# Autodesk Inventor assembly: Motor_ra8846s
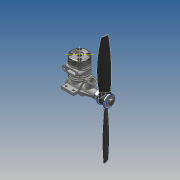
[picture p0: Inventor's stored thumbnail of the model, 180x180]
Saved by Autodesk Inventor 2021 (Build 250183000, 183)
## iProperties
Created: 2021-01-14
Part Number: Motor_ra8846s
Document SubType Name: Assembly
Designer: Sander
Author: Sander
## Documents named in this file (17)
- C:\Users\ricar\OneDrive - Fachhochschule Aachen\Mechatronik I\CAD\INVENTOR\Proyectos\Daten\Motor_ra8846s.iam
- C:\Users\ricar\OneDrive - Fachhochschule Aachen\Mechatronik I\CAD\INVENTOR\Proyectos\Daten\Motorblock_ra8846s.ipt
- C:\Users\ricar\OneDrive - Fachhochschule Aachen\Mechatronik I\CAD\INVENTOR\Proyectos\Daten\Zylinderkopf_ra8846s.ipt
- C:\Users\ricar\OneDrive - Fachhochschule Aachen\Mechatronik I\CAD\INVENTOR\Proyectos\Daten\Gehäusedeckel_ra8846s.ipt
- C:\Users\ricar\OneDrive - Fachhochschule Aachen\Mechatronik I\CAD\INVENTOR\Proyectos\Daten\Zylinderbuchse_ra8846s.ipt
- C:\Users\ricar\OneDrive - Fachhochschule Aachen\Mechatronik I\CAD\INVENTOR\Proyectos\Daten\Zylinderbuchsenring_ra8846s.ipt
- C:\Users\ricar\OneDrive - Fachhochschule Aachen\Mechatronik I\CAD\INVENTOR\Proyectos\Daten\Schlitzschraube_ra8846s\Schlitzschraube_ra8846s-01.ipt
- C:\Users\ricar\OneDrive - Fachhochschule Aachen\Mechatronik I\CAD\INVENTOR\Proyectos\Daten\Schlitzschraube_ra8846s.ipt
- C:\Users\ricar\OneDrive - Fachhochschule Aachen\Mechatronik I\CAD\INVENTOR\Proyectos\Daten\Unterlegescheibe_ra8846s.ipt
- C:\Users\ricar\OneDrive - Fachhochschule Aachen\Mechatronik I\CAD\INVENTOR\Proyectos\Daten\Kurbelwelle_ra8846s.ipt
- C:\Users\ricar\OneDrive - Fachhochschule Aachen\Mechatronik I\CAD\INVENTOR\Proyectos\Daten\Kolben_ra8846s.ipt
- C:\Users\ricar\OneDrive - Fachhochschule Aachen\Mechatronik I\CAD\INVENTOR\Proyectos\Daten\Kolbenbolzen_ra8846s.ipt
- C:\Users\ricar\OneDrive - Fachhochschule Aachen\Mechatronik I\CAD\INVENTOR\Proyectos\Daten\Pleuel_ra8846s.ipt
- C:\Users\ricar\OneDrive - Fachhochschule Aachen\Mechatronik I\CAD\INVENTOR\Proyectos\Daten\Propellernabe_ra8846s.ipt
- C:\Users\ricar\OneDrive - Fachhochschule Aachen\Mechatronik I\CAD\INVENTOR\Proyectos\Daten\propeller_ra8846s.ipt
- C:\Users\ricar\OneDrive - Fachhochschule Aachen\Mechatronik I\CAD\INVENTOR\Proyectos\Daten\Propellerscheib_ra8846s.ipt
- C:\Users\ricar\OneDrive - Fachhochschule Aachen\Mechatronik I\CAD\INVENTOR\Proyectos\Daten\Sechskantenschraube_ra8846s.ipt
## Components (18 placed, 15 different names)
1. Motorblock_ra8846s:1 — Einfügen:1, Einfügen:2, Einfügen:3, Einfügen:4, Einfügen:6, Einfügen:8
2. Zylinderkopf_ra8846s:1 — Einfügen:1, Einfügen:5
3. Gehäusedeckel_ra8846s:1 — Einfügen:2
4. Zylinderbuchse_ra8846s:1 — Einfügen:3, Passend:3
5. Zylinderbuchsenring_ra8846s:1 — Einfügen:4
6. Unterlegescheibe_ra8846s:1 — Einfügen:6, Einfügen:7
7. Kurbelwelle_ra8846s:1 — Einfügen:7, Passend:4
8. Kolben_ra8846s:1 — Passend:1, Passend:2, Passend:3
9. Kolbenbolzen_ra8846s:1 — Passend:1, Passend:2, Passend:5
10. Pleuel_ra8846s:1 — Passend:4, Passend:5
11. Propellernabe_ra8846s:1 — Einfügen:8, Einfügen:9
12. propeller_ra8846s:1 — Einfügen:9, Passend:6
13. Propellerscheib_ra8846s:1 — Passend:6, Einfügen:10
14. Sechskantenschraube_ra8846s:1 — Einfügen:10
15. Schlitzschraube_ra8846s-01:1 — Einfügen:5
16. Schlitzschraube_ra8846s-01:2
17. Schlitzschraube_ra8846s-01:3
18. Schlitzschraube_ra8846s-01:4
## Component patterns: (4 elements, first: Schlitzschraube_ra8846s-01:1)
## Relationships (16: Insert 10, Mate 6)
- Einfügen:1 [Insert]: Motorblock_ra8846s:1 ↔ Zylinderkopf_ra8846s:1
- Einfügen:2 [Insert]: Motorblock_ra8846s:1 ↔ Gehäusedeckel_ra8846s:1
- Einfügen:3 [Insert]: Motorblock_ra8846s:1 ↔ Zylinderbuchse_ra8846s:1
- Einfügen:4 [Insert]: Motorblock_ra8846s:1 ↔ Zylinderbuchsenring_ra8846s:1
- Einfügen:5 [Insert]: Zylinderkopf_ra8846s:1 ↔ Schlitzschraube_ra8846s-01:1
- Einfügen:6 [Insert]: Motorblock_ra8846s:1 ↔ Unterlegescheibe_ra8846s:1
- Einfügen:7 [Insert]: Unterlegescheibe_ra8846s:1 ↔ Kurbelwelle_ra8846s:1
- Passend:1 [Mate]: Kolben_ra8846s:1 ↔ Kolbenbolzen_ra8846s:1
- Passend:2 [Mate] (-6 mm): Kolben_ra8846s:1 ↔ Kolbenbolzen_ra8846s:1
- Passend:3 [Mate]: Zylinderbuchse_ra8846s:1 ↔ Kolben_ra8846s:1
- Passend:4 [Mate]: Kurbelwelle_ra8846s:1 ↔ Pleuel_ra8846s:1
- Passend:5 [Mate]: Kolbenbolzen_ra8846s:1 ↔ Pleuel_ra8846s:1
- Einfügen:8 [Insert]: Motorblock_ra8846s:1 ↔ Propellernabe_ra8846s:1
- Einfügen:9 [Insert] (0.17 mm): Propellernabe_ra8846s:1 ↔ propeller_ra8846s:1
- Passend:6 [Mate]: propeller_ra8846s:1 ↔ Propellerscheib_ra8846s:1
- Einfügen:10 [Insert]: Propellerscheib_ra8846s:1 ↔ Sechskantenschraube_ra8846s:1
